# Autodesk Inventor assembly: Joint Assembly
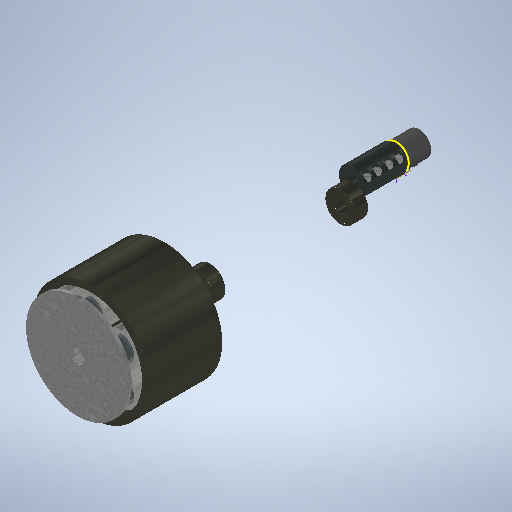
[picture p0: Inventor's stored thumbnail of the model, 512x512]
Saved by Autodesk Inventor 2025 (Build 290162000, 162)
## iProperties
Created: 2026-07-22
Part Number: Joint Assembly
Document SubType Name: Assembly
Designer: matot
Author: matot
## Documents named in this file (7)
- C:\Users\matot\OneDrive - Stellenbosch University\2026\MechatronicsProject478\Building the joint\Joint Assembly\Joint Assembly.iam
- C:\Users\matot\OneDrive - Stellenbosch University\2026\MechatronicsProject478\Building the joint\Joint Assembly\Brake disc.ipt
- C:\Users\matot\OneDrive - Stellenbosch University\2026\MechatronicsProject478\Building the joint\Joint Assembly\Electromagnet.iam
- C:\Users\matot\OneDrive - Stellenbosch University\2026\MechatronicsProject478\Building the joint\Joint Assembly\2058786.iam
- C:\Users\matot\OneDrive - Stellenbosch University\2026\MechatronicsProject478\Building the joint\Joint Assembly\mclx-20-20-f.iam
- C:\Users\matot\OneDrive - Stellenbosch University\2026\MechatronicsProject478\Building the joint\Joint Assembly\Reducer bushing.ipt
- C:\Users\matot\OneDrive - Stellenbosch University\2026\MechatronicsProject478\Building the joint\Joint Assembly\Optical Encoder.ipt
## Components (7 placed, 6 different names)
1. Brake disc:1
2. Electromagnet:1 [sub-assembly]
3. 2058786:1 [sub-assembly]
4. 2058786:2 [sub-assembly]
5. mclx-20-20-f:1 [sub-assembly] — Insert:1
6. Reducer bushing:2 — Insert:1, Insert:2
7. Optical Encoder:1 — Insert:2
## Relationships (2: Insert 2)
- Insert:1: mclx-20-20-f:1 ↔ Reducer bushing:2
- Insert:2: Reducer bushing:2 ↔ Optical Encoder:1
